# Autodesk Inventor assembly: A2017_T2_09
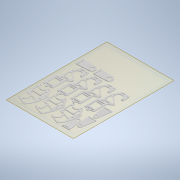
[picture p0: Inventor's stored thumbnail of the model, 180x180]
Saved by Autodesk Inventor 2020 (Build 240168000, 168)
## iProperties
Created: 2021-08-27
Part Number: A2017_T2_09
Document SubType Name: Assembly
Designer: Masato
Author: Masato
## Documents named in this file (6)
- C:\Inventor\SUSTAINA-OP\Cam\A2017_T2_09.iam
- C:\Inventor\SUSTAINA-OP\Cam\DisposableBoard.ipt
- C:\Inventor\SUSTAINA-OP\LowerBody\Knee\Knee_side_frame.ipt
- C:\Inventor\SUSTAINA-OP\LowerBody\Ankle\Ankle_side_frame.ipt
- C:\Inventor\SUSTAINA-OP\LowerBody\Foot\Foot_front_frame.ipt
- C:\Inventor\SUSTAINA-OP\LowerBody\Foot\Foot_back_frame.ipt
## Components (13 placed, 5 different names)
1. DisposableBoard:1 — メイト:2, メイト:1, フラッシュ:1, フラッシュ:2, メイト:4, フラッシュ:3, 正接:1, メイト:5, メイト:6, フラッシュ:4, メイト:7, フラッシュ:5, フラッシュ:6, メイト:10, フラッシュ:7
2. Foot_front_frame:1 — メイト:6, フラッシュ:4, 正接:2, メイト:8
3. Knee_side_frame:1 — メイト:4, フラッシュ:3, 正接:1, メイト:9
4. Knee_side_frame:2
5. Knee_side_frame:3 — 正接:2
6. Ankle_side_frame:2 — メイト:5, フラッシュ:6, メイト:9, 正接:3
7. Ankle_side_frame:3
8. Ankle_side_frame:4
9. Ankle_side_frame:5
10. Foot_front_frame:2 — メイト:7, メイト:8, フラッシュ:5
11. Foot_front_frame:3
12. Foot_back_frame:1 — メイト:10, フラッシュ:7, 正接:3
13. Foot_back_frame:2
## Component patterns: (3 elements, first: Knee_side_frame:1), (4 elements, first: Ankle_side_frame:2), (2 elements, first: Foot_front_frame:2), (2 elements, first: Foot_back_frame:1)
## Relationships (19: Mate 9, Flush 7, Tangent 3)
- メイト:2 [Mate]: DisposableBoard:1
- メイト:1 [Mate]: DisposableBoard:1
- フラッシュ:1 [Flush]: DisposableBoard:1
- フラッシュ:2 [Flush]: DisposableBoard:1
- メイト:4 [Mate]: DisposableBoard:1 ↔ Knee_side_frame:1
- フラッシュ:3 [Flush] (2 mm): DisposableBoard:1 ↔ Knee_side_frame:1
- 正接:1 [Tangent] (2 mm): DisposableBoard:1 ↔ Knee_side_frame:1
- メイト:5 [Mate]: DisposableBoard:1 ↔ Ankle_side_frame:2
- メイト:6 [Mate]: DisposableBoard:1 ↔ Foot_front_frame:1
- フラッシュ:4 [Flush] (2 mm): DisposableBoard:1 ↔ Foot_front_frame:1
- 正接:2 [Tangent] (2.5 mm): Foot_front_frame:1 ↔ Knee_side_frame:3
- メイト:7 [Mate]: DisposableBoard:1 ↔ Foot_front_frame:2
- メイト:8 [Mate] (2.5 mm): Foot_front_frame:1 ↔ Foot_front_frame:2
- フラッシュ:5 [Flush] (2 mm): DisposableBoard:1 ↔ Foot_front_frame:2
- フラッシュ:6 [Flush] (2 mm): DisposableBoard:1 ↔ Ankle_side_frame:2
- メイト:9 [Mate] (2.5 mm): Knee_side_frame:1 ↔ Ankle_side_frame:2
- メイト:10 [Mate]: DisposableBoard:1 ↔ Foot_back_frame:1
- フラッシュ:7 [Flush] (2 mm): DisposableBoard:1 ↔ Foot_back_frame:1
- 正接:3 [Tangent] (5.5 mm): Ankle_side_frame:2 ↔ Foot_back_frame:1
